# Autodesk Inventor assembly: BackLiftProto
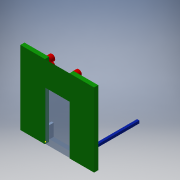
[picture p0: Inventor's stored thumbnail of the model, 180x180]
Saved by Autodesk Inventor 2017 (Build 210142000, 142)
## iProperties
Created: 2017-11-11
Part Number: BackLiftProto
Document SubType Name: Assembly
Designer: User
Author: User
## Documents named in this file (5)
- C:\Robotics\CAD\2017-18_CAD\Prototypes\BackLiftProto.iam
- C:\Robotics\CAD\2017-18_CAD\Prototypes\BackLiftProtoPart3.ipt
- C:\Robotics\CAD\2017-18_CAD\Prototypes\BackLiftProtoPart4.ipt
- C:\Robotics\CAD\2017-18_CAD\Prototypes\BackLiftProtoPart6.ipt
- C:\Robotics\CAD\2017-18_CAD\Prototypes\BackLiftProtoPart7.ipt
## Components (9 placed, 4 different names)
1. BackLiftProtoPart3:1 — Flush:4, Flush:5, Mate:1, Tangent:1, Tangent:2, Tangent:3, Mate:2, Tangent:4, Mate:3, Tangent:6, Tangent:8, Tangent:10, Tangent:12
2. BackLiftProtoPart4:1 — Flush:4, Flush:5, Flush:6, Mate:4
3. BackLiftProtoPart6:1 — Mate:1, Tangent:1, Tangent:2, Tangent:5, Flush:7
4. BackLiftProtoPart6:2 — Tangent:3, Mate:2, Tangent:4, Flush:9, Flush:10, Tangent:9
5. BackLiftProtoPart7:1 — Mate:3, Flush:6, Mate:4
6. BackLiftProtoPart6:3 — Flush:9, Tangent:11, Tangent:12
7. BackLiftProtoPart6:4 — Flush:10, Tangent:9, Tangent:10, Tangent:11
8. BackLiftProtoPart6:5 — Tangent:5, Flush:7, Tangent:6, Flush:8, Tangent:7
9. BackLiftProtoPart6:6 — Flush:8, Tangent:7, Tangent:8
## Relationships (23: Tangent 12, Flush 7, Mate 4)
- Flush:4: BackLiftProtoPart3:1 ↔ BackLiftProtoPart4:1
- Flush:5 (152.4 mm): BackLiftProtoPart3:1 ↔ BackLiftProtoPart4:1
- Mate:1: BackLiftProtoPart3:1 ↔ BackLiftProtoPart6:1
- Tangent:1: BackLiftProtoPart3:1 ↔ BackLiftProtoPart6:1
- Tangent:2 (-25.4 mm): BackLiftProtoPart3:1 ↔ BackLiftProtoPart6:1
- Tangent:3: BackLiftProtoPart3:1 ↔ BackLiftProtoPart6:2
- Mate:2: BackLiftProtoPart3:1 ↔ BackLiftProtoPart6:2
- Tangent:4 (-25.4 mm): BackLiftProtoPart3:1 ↔ BackLiftProtoPart6:2
- Mate:3: BackLiftProtoPart3:1 ↔ BackLiftProtoPart7:1
- Flush:6: BackLiftProtoPart4:1 ↔ BackLiftProtoPart7:1
- Mate:4: BackLiftProtoPart4:1 ↔ BackLiftProtoPart7:1
- Tangent:5: BackLiftProtoPart6:1 ↔ BackLiftProtoPart6:5
- Flush:7: BackLiftProtoPart6:1 ↔ BackLiftProtoPart6:5
- Tangent:6 (-25.4 mm): BackLiftProtoPart3:1 ↔ BackLiftProtoPart6:5
- Flush:8: BackLiftProtoPart6:5 ↔ BackLiftProtoPart6:6
- Tangent:7: BackLiftProtoPart6:5 ↔ BackLiftProtoPart6:6
- Tangent:8 (-25.4 mm): BackLiftProtoPart3:1 ↔ BackLiftProtoPart6:6
- Flush:9: BackLiftProtoPart6:2 ↔ BackLiftProtoPart6:3
- Flush:10: BackLiftProtoPart6:2 ↔ BackLiftProtoPart6:4
- Tangent:9: BackLiftProtoPart6:2 ↔ BackLiftProtoPart6:4
- Tangent:10 (-25.4 mm): BackLiftProtoPart3:1 ↔ BackLiftProtoPart6:4
- Tangent:11: BackLiftProtoPart6:3 ↔ BackLiftProtoPart6:4
- Tangent:12 (-25.4 mm): BackLiftProtoPart3:1 ↔ BackLiftProtoPart6:3
